# Autodesk Inventor assembly: Assembly1
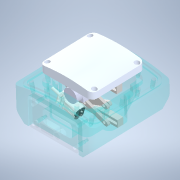
[picture p0: Inventor's stored thumbnail of the model, 180x180]
Saved by Autodesk Inventor 2020.1 (Build 241239000, 239)
## iProperties
Created: 2019-10-17
Part Number: Assembly1
Document SubType Name: Assembly
Designer: jesse
Author: jesse
## Documents named in this file (7)
- C:\Users\jesse\Desktop\rocksat_2020_model\Assembly1.iam
- C:\Users\jesse\Desktop\rocksat_2020_model\MultipurposePort-Released_withSTL\Assembly Multipurpose Port.iam
- C:\Users\jesse\Desktop\rocksat_2020_model\n20-micro-metal-gearmotor-1.snapshot.2\n20 motor.iam
- C:\Users\jesse\Desktop\rocksat_2020_model\camera.ipt
- C:\Users\jesse\Desktop\rocksat_2020_model\s_arm.ipt
- C:\Users\jesse\Desktop\rocksat_2020_model\s_support.ipt
- C:\Users\jesse\Desktop\rocksat_2020_model\MultipurposePort-Released_withSTL\ME112673.ipt
## Components (11 placed, 6 different names)
1. Assembly Multipurpose Port:1 [sub-assembly] — Mate:1, Mate:2, Flush:1, Flush:2, Mate:5, Mate:11, Mate:12, Mate:15
2. n20 motor:1 [sub-assembly] — Mate:1, Mate:2
3. camera:1 — Mate:13, Flush:5, Flush:6, Flush:7
4. s_arm:1 — Rotational:1, Tangent:1, Mate:3, Mate:6
5. s_arm:2 — Rotational:1, Rotational:2, Mate:7, Mate:8
6. s_support:1 — Flush:1, Flush:2, Rotational:2, Tangent:1, Mate:3, Flush:3, Flush:4, Mate:5
7. s_support:3 — Flush:3, Flush:4, Mate:9, Mate:10
8. s_arm:3 — Mate:6
9. s_arm:4 — Mate:7, Mate:8, Mate:9
10. ME112673:1 — Mate:10, Mate:11, Mate:12, Mate:13, Flush:5, Flush:6, Mate:14, Flush:8, Mate:15
11. camera:2 — Mate:14, Flush:7, Flush:8
## Relationships (26: Mate 14, Flush 8, RevoluteJoint 3, Tangent 1)
- Mate:1: Assembly Multipurpose Port:1 ↔ n20 motor:1
- Mate:2: Assembly Multipurpose Port:1 ↔ n20 motor:1
- Rotational:1 [RevoluteJoint]: s_arm:1 ↔ s_arm:2
- Flush:1: Assembly Multipurpose Port:1 ↔ s_support:1
- Flush:2: Assembly Multipurpose Port:1 ↔ s_support:1
- Rotational:2 [RevoluteJoint]: s_arm:2 ↔ s_support:1
- Tangent:1: s_arm:1 ↔ s_support:1
- Mate:3: s_arm:1 ↔ s_support:1
- Flush:3: s_support:1 ↔ s_support:3
- Flush:4: s_support:1 ↔ s_support:3
- Mate:5: Assembly Multipurpose Port:1 ↔ s_support:1
- [RevoluteJoint]: s_arm:3 ↔ s_arm:4
- Mate:6: s_arm:1 ↔ s_arm:3
- Mate:7: s_arm:2 ↔ s_arm:4
- Mate:8: s_arm:2 ↔ s_arm:4
- Mate:9: s_support:3 ↔ s_arm:4
- Mate:10: s_support:3 ↔ ME112673:1
- Mate:11: Assembly Multipurpose Port:1 ↔ ME112673:1
- Mate:12: Assembly Multipurpose Port:1 ↔ ME112673:1
- Mate:13: camera:1 ↔ ME112673:1
- Flush:5: camera:1 ↔ ME112673:1
- Flush:6 (-29.0068 mm): camera:1 ↔ ME112673:1
- Mate:14: ME112673:1 ↔ camera:2
- Flush:7: camera:1 ↔ camera:2
- Flush:8: ME112673:1 ↔ camera:2
- Mate:15: Assembly Multipurpose Port:1 ↔ ME112673:1
## Named parameters: support_length = 58.42 mm, s_arm_length = 58.42 mm, d17_d2 = 0 mm, d18_d3 = 138.35825 deg
